# Autodesk Inventor assembly: 振動ナイフモデル
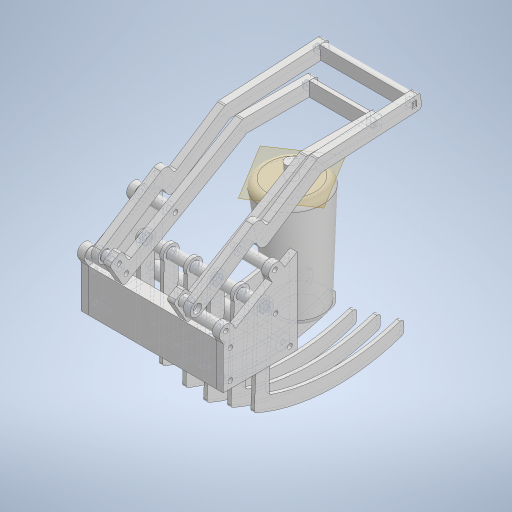
[picture p0: Inventor's stored thumbnail of the model, 512x512]
Saved by Autodesk Inventor 2024.3 (Build 283343000, 343)
## iProperties
Created: 2024-10-09
Part Number: 振動ナイフモデル
Document SubType Name: Assembly
Designer: hikou
Author: hikou
## Documents named in this file (17)
- C:\Users\hikou\OneDrive\ドキュメント\Inventor\end_effector\harvesting_endeffector\Vibrating_knife_endeffector\model\振動ナイフモデル.iam
- C:\Users\hikou\OneDrive\ドキュメント\Inventor\end_effector\harvesting_endeffector\Vibrating_knife_endeffector\model\茎固定パーツ.ipt
- C:\Users\hikou\OneDrive\ドキュメント\Inventor\end_effector\harvesting_endeffector\Vibrating_knife_endeffector\model\茎固定パーツ2.ipt
- C:\Users\hikou\OneDrive\ドキュメント\Inventor\end_effector\harvesting_endeffector\Vibrating_knife_endeffector\model\ベースパーツ.ipt
- C:\Users\hikou\OneDrive\ドキュメント\Inventor\end_effector\harvesting_endeffector\Vibrating_knife_endeffector\model\ベースパーツ_アーム固定部分.ipt
- C:\Users\hikou\OneDrive\ドキュメント\Inventor\end_effector\harvesting_endeffector\Vibrating_knife_endeffector\model\ベースパーツ_実験装置取り付け部分.ipt
- C:\Users\hikou\OneDrive\ドキュメント\Inventor\end_effector\harvesting_endeffector\Vibrating_knife_endeffector\model\刃固定パーツ.ipt
- C:\Users\hikou\OneDrive\ドキュメント\Inventor\end_effector\harvesting_endeffector\Vibrating_knife_endeffector\model\刃.ipt
- C:\Users\hikou\OneDrive\ドキュメント\Inventor\end_effector\harvesting_endeffector\Vibrating_knife_endeffector\model\スペーサ4.4mm_内径3.3mm.ipt
- C:\Users\hikou\OneDrive\ドキュメント\Inventor\end_effector\harvesting_endeffector\Vibrating_knife_endeffector\model\ベアリング.ipt
- C:\Users\hikou\OneDrive\ドキュメント\Inventor\end_effector\harvesting_endeffector\Vibrating_knife_endeffector\model\指_大.ipt
- C:\Users\hikou\OneDrive\ドキュメント\Inventor\end_effector\harvesting_endeffector\Vibrating_knife_endeffector\model\スペーサ7mm_内径3.3mm.ipt
- C:\Users\hikou\OneDrive\ドキュメント\Inventor\end_effector\harvesting_endeffector\Vibrating_knife_endeffector\model\指_中.ipt
- C:\Users\hikou\OneDrive\ドキュメント\Inventor\end_effector\harvesting_endeffector\Vibrating_knife_endeffector\model\指_小.ipt
- C:\Users\hikou\OneDrive\ドキュメント\Inventor\end_effector\harvesting_endeffector\Vibrating_knife_endeffector\model\簡易ピーマン.ipt
- C:\Users\hikou\OneDrive\ドキュメント\Inventor\end_effector\harvesting_endeffector\Vibrating_knife_endeffector\model\スペーサ20mm_内径3.3mm.ipt
- C:\Users\hikou\OneDrive\ドキュメント\Inventor\end_effector\harvesting_endeffector\Vibrating_knife_endeffector\model\スペーサ2.5mm_内径3.3mm.ipt
## Components (38 placed, 16 different names)
1. 茎固定パーツ:1 — メイト:4, メイト:5, メイト:6, 挿入:13
2. 茎固定パーツ:2 — メイト:1, メイト:2, メイト:3, 挿入:12
3. 茎固定パーツ2:1 — メイト:1, メイト:2, メイト:3, メイト:4, メイト:5, メイト:6
4. ベースパーツ:1 — 挿入:1, 挿入:36, 挿入:43, 挿入:44, 挿入:48, 挿入:49
5. ベースパーツ:2 — 挿入:2, 挿入:4, 挿入:5, 挿入:37, 挿入:38, 挿入:46
6. ベースパーツ_アーム固定部分:1 — 挿入:1, 挿入:2, 挿入:5
7. ベースパーツ_実験装置取り付け部分:1 — 挿入:4, メイト:7, 挿入:36, 挿入:49
8. 刃固定パーツ:1 — メイト:8, メイト:9, メイト:10, 挿入:41, 挿入:42
9. 刃固定パーツ:2 — メイト:11, メイト:12, メイト:13, 挿入:16, 挿入:39, 挿入:40
10. 刃:1 — メイト:8, メイト:9, メイト:10, メイト:11, メイト:12, メイト:13
11. スペーサ4.4mm_内径3.3mm:1 — 挿入:15, 挿入:16
12. スペーサ4.4mm_内径3.3mm:2 — 挿入:14
13. ベアリング:1 — 挿入:12, 挿入:15
14. ベアリング:2 — 挿入:13, 挿入:14
15. 指_大:1 — 挿入:17
16. 指_大:2 — 挿入:18
17. ベアリング:3 — 挿入:23, 挿入:25, 挿入:27
18. ベアリング:4 — 挿入:24, 挿入:26, 挿入:28
19. ベアリング:5 — 挿入:29, 挿入:31, 挿入:47
20. ベアリング:6 — 挿入:18, 挿入:20, 挿入:22
21. ベアリング:7 — 挿入:17, 挿入:19, 挿入:21
22. ベアリング:8 — 挿入:30, 挿入:32, 挿入:45
23. スペーサ7mm_内径3.3mm:1 — 挿入:27, 挿入:31
24. スペーサ7mm_内径3.3mm:2 — 挿入:28, 挿入:32
25. スペーサ7mm_内径3.3mm:3 — 挿入:21, 挿入:25
26. スペーサ7mm_内径3.3mm:4 — 挿入:22, 挿入:26
27. スペーサ7mm_内径3.3mm:5 — 挿入:19, 挿入:20
28. 指_中:1 — 挿入:23
29. 指_中:2 — 挿入:24
30. 指_小:1 — 挿入:29
31. 指_小:2 — 挿入:30
32. 簡易ピーマン:1
33. スペーサ20mm_内径3.3mm:1 — 挿入:41, 挿入:44
34. スペーサ20mm_内径3.3mm:2 — 挿入:42, 挿入:43
35. スペーサ20mm_内径3.3mm:3 — 挿入:38, 挿入:40
36. スペーサ20mm_内径3.3mm:4 — 挿入:37, 挿入:39
37. スペーサ2.5mm_内径3.3mm:1 — 挿入:47, 挿入:48
38. スペーサ2.5mm_内径3.3mm:2 — 挿入:45, 挿入:46
## Relationships (52: Insert 39, Mate 13)
- メイト:1 [Mate]: 茎固定パーツ:2 ↔ 茎固定パーツ2:1
- メイト:2 [Mate]: 茎固定パーツ:2 ↔ 茎固定パーツ2:1
- メイト:3 [Mate]: 茎固定パーツ:2 ↔ 茎固定パーツ2:1
- メイト:4 [Mate]: 茎固定パーツ:1 ↔ 茎固定パーツ2:1
- メイト:5 [Mate]: 茎固定パーツ:1 ↔ 茎固定パーツ2:1
- メイト:6 [Mate]: 茎固定パーツ:1 ↔ 茎固定パーツ2:1
- 挿入:1 [Insert]: ベースパーツ:1 ↔ ベースパーツ_アーム固定部分:1
- 挿入:2 [Insert]: ベースパーツ:2 ↔ ベースパーツ_アーム固定部分:1
- 挿入:4 [Insert]: ベースパーツ:2 ↔ ベースパーツ_実験装置取り付け部分:1
- メイト:7 [Mate]: ベースパーツ_実験装置取り付け部分:1
- 挿入:5 [Insert]: ベースパーツ:2 ↔ ベースパーツ_アーム固定部分:1
- メイト:8 [Mate]: 刃固定パーツ:1 ↔ 刃:1
- メイト:9 [Mate]: 刃固定パーツ:1 ↔ 刃:1
- メイト:10 [Mate]: 刃固定パーツ:1 ↔ 刃:1
- メイト:11 [Mate]: 刃固定パーツ:2 ↔ 刃:1
- メイト:12 [Mate]: 刃固定パーツ:2 ↔ 刃:1
- メイト:13 [Mate]: 刃固定パーツ:2 ↔ 刃:1
- 挿入:12 [Insert]: 茎固定パーツ:2 ↔ ベアリング:1
- 挿入:13 [Insert]: 茎固定パーツ:1 ↔ ベアリング:2
- 挿入:14 [Insert]: スペーサ4.4mm_内径3.3mm:2 ↔ ベアリング:2
- 挿入:15 [Insert]: スペーサ4.4mm_内径3.3mm:1 ↔ ベアリング:1
- 挿入:16 [Insert]: 刃固定パーツ:2 ↔ スペーサ4.4mm_内径3.3mm:1
- 挿入:17 [Insert]: 指_大:1 ↔ ベアリング:7
- 挿入:18 [Insert]: 指_大:2 ↔ ベアリング:6
- 挿入:19 [Insert]: ベアリング:7 ↔ スペーサ7mm_内径3.3mm:5
- 挿入:20 [Insert]: ベアリング:6 ↔ スペーサ7mm_内径3.3mm:5
- 挿入:21 [Insert]: ベアリング:7 ↔ スペーサ7mm_内径3.3mm:3
- 挿入:22 [Insert]: ベアリング:6 ↔ スペーサ7mm_内径3.3mm:4
- 挿入:23 [Insert]: ベアリング:3 ↔ 指_中:1
- 挿入:24 [Insert]: ベアリング:4 ↔ 指_中:2
- 挿入:25 [Insert]: ベアリング:3 ↔ スペーサ7mm_内径3.3mm:3
- 挿入:26 [Insert]: ベアリング:4 ↔ スペーサ7mm_内径3.3mm:4
- 挿入:27 [Insert]: ベアリング:3 ↔ スペーサ7mm_内径3.3mm:1
- 挿入:28 [Insert]: ベアリング:4 ↔ スペーサ7mm_内径3.3mm:2
- 挿入:29 [Insert]: ベアリング:5 ↔ 指_小:1
- 挿入:30 [Insert]: ベアリング:8 ↔ 指_小:2
- 挿入:31 [Insert]: ベアリング:5 ↔ スペーサ7mm_内径3.3mm:1
- 挿入:32 [Insert]: ベアリング:8 ↔ スペーサ7mm_内径3.3mm:2
- 挿入:36 [Insert]: ベースパーツ:1 ↔ ベースパーツ_実験装置取り付け部分:1
- 挿入:37 [Insert]: ベースパーツ:2 ↔ スペーサ20mm_内径3.3mm:4
- 挿入:38 [Insert]: ベースパーツ:2 ↔ スペーサ20mm_内径3.3mm:3
- 挿入:39 [Insert]: 刃固定パーツ:2 ↔ スペーサ20mm_内径3.3mm:4
- 挿入:40 [Insert]: 刃固定パーツ:2 ↔ スペーサ20mm_内径3.3mm:3
- 挿入:41 [Insert]: 刃固定パーツ:1 ↔ スペーサ20mm_内径3.3mm:1
- 挿入:42 [Insert]: 刃固定パーツ:1 ↔ スペーサ20mm_内径3.3mm:2
- 挿入:43 [Insert]: ベースパーツ:1 ↔ スペーサ20mm_内径3.3mm:2
- 挿入:44 [Insert]: ベースパーツ:1 ↔ スペーサ20mm_内径3.3mm:1
- 挿入:45 [Insert]: ベアリング:8 ↔ スペーサ2.5mm_内径3.3mm:2
- 挿入:46 [Insert]: ベースパーツ:2 ↔ スペーサ2.5mm_内径3.3mm:2
- 挿入:47 [Insert]: ベアリング:5 ↔ スペーサ2.5mm_内径3.3mm:1
- 挿入:48 [Insert]: ベースパーツ:1 ↔ スペーサ2.5mm_内径3.3mm:1
- 挿入:49 [Insert]: ベースパーツ:1 ↔ ベースパーツ_実験装置取り付け部分:1
